# Autodesk Inventor assembly: ensamble_griper
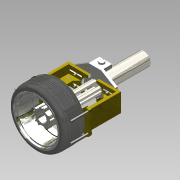
[picture p0: Inventor's stored thumbnail of the model, 180x180]
Saved by Autodesk Inventor 2021 (Build 250183000, 183)
## iProperties
Created: 2022-01-31
Part Number: ensamble_griper
Document SubType Name: Assembly
Designer: Osmar Ediber Toloza Bernal
Mass: 94323.7 g
Surface Area: 50929.7 cm^2
Volume: 46606.4 cm^3
Density: 2.02383 g/cm^3
Author: Osmar Ediber Toloza Bernal
## Documents named in this file (6)
- H:\Mi unidad\2021 2\Robotica\Proyecto\modelado\griper\ensamble_griper.iam
- H:\Mi unidad\2021 2\Robotica\Proyecto\modelado\griper\soporte.ipt
- H:\Mi unidad\2021 2\Robotica\Proyecto\modelado\griper\garra_griper.ipt
- H:\Mi unidad\2021 2\Robotica\Proyecto\modelado\griper\garra_griper_MIR.ipt
- H:\Mi unidad\2021 2\Robotica\Proyecto\modelado\griper\llanta\lancerwheel.iam
- H:\Mi unidad\2021 2\Robotica\Proyecto\modelado\griper\atornillador.ipt
## Components (5 placed, 5 different names)
1. soporte:1 — Nivelación:1, Coincidencia:1, Coincidencia:2, Tangente:1, Coincidencia:4, Tangente:2, Coincidencia:5, Tangente:3, Tangente:4, Coincidencia:6, Rígido:1
2. garra_griper:1 — Tangente:1, Coincidencia:5, Tangente:3, Coincidencia:6
3. garra_griper_MIR:1 — Coincidencia:4, Tangente:2, Tangente:4
4. atornillador:1 — Rígido:1, Insertar:1, Insertar:2
5. lancerwheel:1 [sub-assembly] — Insertar:1, Insertar:2
## Relationships (13: Mate 5, Tangent 4, Insert 2, Flush 1, WeldJoint 1)
- Nivelación:1 [Flush]: soporte:1
- Coincidencia:1 [Mate]: soporte:1
- Coincidencia:2 [Mate]: soporte:1
- Tangente:1: soporte:1 ↔ garra_griper:1
- Coincidencia:4 [Mate]: soporte:1 ↔ garra_griper_MIR:1
- Tangente:2: soporte:1 ↔ garra_griper_MIR:1
- Coincidencia:5 [Mate]: soporte:1 ↔ garra_griper:1
- Tangente:3: soporte:1 ↔ garra_griper:1
- Tangente:4: soporte:1 ↔ garra_griper_MIR:1
- Coincidencia:6 [Mate]: soporte:1 ↔ garra_griper:1
- Rígido:1 [WeldJoint]: soporte:1 ↔ atornillador:1
- Insertar:1: atornillador:1 ↔ lancerwheel:1
- Insertar:2: atornillador:1 ↔ lancerwheel:1
